# Autodesk Inventor assembly: 頭_1_2
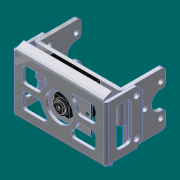
[picture p0: Inventor's stored thumbnail of the model, 180x180]
Saved by Autodesk Inventor 2016 (Build 200138000, 138)
## iProperties
Created: 2016-05-10
Part Number: 頭_1_2
Document SubType Name: Assembly
Designer: hiroaki
Mass: 17.9103 g
Surface Area: 119.086 cm^2
Volume: 7.5268 cm^3
Density: 2.37954 g/cm^3
Author: hiroaki
## Documents named in this file (5)
- C:\Users\hiro\Documents\kenkyuu\二足\二足ver6.0\上半身\頭\頭_1_2.iam
- C:\Users\hiro\Documents\kenkyuu\二足\二足ver6.0\上半身\頭\頭_メインフレーム_1_2.ipt
- C:\Users\hiro\Documents\kenkyuu\二足\二足ver6.0\インポートされたコンポーネント\RasPi_Camera\RasPi_Camera.iam
- C:\Users\hiro\Documents\kenkyuu\二足\二足ver6.0\上半身\頭\頭_メインフレーム_1_3.ipt
- C:\Users\hiro\Documents\kenkyuu\二足\二足ver6.0\上半身\頭\頭_メインフレーム_1_4.ipt
## Components (4 placed, 4 different names)
1. 頭_メインフレーム_1_2:1 — 挿入:1, 挿入:2, メイト:4, メイト:5, メイト:6
2. RasPi_Camera:1 [sub-assembly] — 挿入:3, 挿入:4, 挿入:5
3. 頭_メインフレーム_1_3:1 — 挿入:1, 挿入:2, 挿入:3, 挿入:4, 挿入:5, メイト:1, メイト:2, フラッシュ:1
4. 頭_メインフレーム_1_4:1 — メイト:4, メイト:5, メイト:6
## Relationships (11: Insert 5, Mate 5, Flush 1)
- 挿入:1 [Insert]: 頭_メインフレーム_1_2:1 ↔ 頭_メインフレーム_1_3:1
- 挿入:2 [Insert]: 頭_メインフレーム_1_2:1 ↔ 頭_メインフレーム_1_3:1
- 挿入:3 [Insert]: RasPi_Camera:1 ↔ 頭_メインフレーム_1_3:1
- 挿入:4 [Insert]: RasPi_Camera:1 ↔ 頭_メインフレーム_1_3:1
- 挿入:5 [Insert]: RasPi_Camera:1 ↔ 頭_メインフレーム_1_3:1
- メイト:1 [Mate]: 頭_メインフレーム_1_3:1
- メイト:2 [Mate]: 頭_メインフレーム_1_3:1
- フラッシュ:1 [Flush]: 頭_メインフレーム_1_3:1
- メイト:4 [Mate]: 頭_メインフレーム_1_2:1 ↔ 頭_メインフレーム_1_4:1
- メイト:5 [Mate]: 頭_メインフレーム_1_2:1 ↔ 頭_メインフレーム_1_4:1
- メイト:6 [Mate]: 頭_メインフレーム_1_2:1 ↔ 頭_メインフレーム_1_4:1
